# Autodesk Inventor assembly: asiyunit
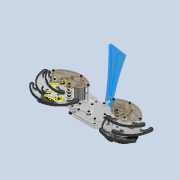
[picture p0: Inventor's stored thumbnail of the model, 180x180]
Saved by Autodesk Inventor 2020.4 (Build 244396000, 396)
## iProperties
Created: 2021-02-23
Part Number: asiyunit
Document SubType Name: Assembly
Designer: AA19065
Mass: 835.935 g
Surface Area: 3123.14 cm^2
Volume: 276.7 cm^3
Density: 3.02108 g/cm^3
Author: AA19065
## Documents named in this file (24)
- C:\Users\happy\OneDrive\ドキュメント\賢一ファイル\SRDC\試作10-2\アセンブリ\脚ユニット.iam
- C:\Users\happy\OneDrive\ドキュメント\賢一ファイル\SRDC\試作10-2\アセンブリ\前足.iam
- C:\Users\happy\OneDrive\ドキュメント\賢一ファイル\SRDC\試作10-2\アセンブリ\M-前足.iam
- C:\Users\happy\OneDrive\ドキュメント\賢一ファイル\SRDC\試作10-2\フレーム\脚中間フレーム内v2.ipt
- C:\Users\happy\OneDrive\ドキュメント\賢一ファイル\SRDC\試作10-2\フレーム\脚中間フレーム外v2.ipt
- C:\Users\happy\OneDrive\ドキュメント\賢一ファイル\SRDC\試作10-2\スペーサ\5mm.ipt
- C:\Users\happy\OneDrive\ドキュメント\賢一ファイル\SRDC\試作10-2\ねじ\m3皿ネジ5 (1).ipt
- C:\Users\happy\OneDrive\ドキュメント\賢一ファイル\SRDC\試作10-2\フレーム\アンノーン後.ipt
- C:\Users\happy\OneDrive\ドキュメント\賢一ファイル\SRDC\試作10-2\フレーム\アンノーン前.ipt
- C:\Users\happy\OneDrive\ドキュメント\賢一ファイル\SRDC\試作10-2\スペーサ\12mm.ipt
- C:\Users\happy\OneDrive\ドキュメント\賢一ファイル\SRDC\試作10-2\ねじ\M3ボタンボルト8.ipt
- C:\Users\happy\OneDrive\ドキュメント\賢一ファイル\SRDC\試作10-2\フレーム\heiko-ue.ipt
- C:\Users\happy\OneDrive\ドキュメント\賢一ファイル\SRDC\試作10-2\フレーム\hieko-sita.ipt
- C:\Users\happy\OneDrive\ドキュメント\賢一ファイル\SRDC\試作10-2\軸受け\オイレスw3f6-8a.ipt
- C:\Users\happy\OneDrive\ドキュメント\賢一ファイル\SRDC\試作10-2\軸受け\オイレスw1.5f6-8n.ipt
- C:\Users\happy\OneDrive\ドキュメント\賢一ファイル\SRDC\試作10-2\ねじ\ワッシャ3-8  0.5.ipt
- C:\Users\happy\OneDrive\ドキュメント\賢一ファイル\SRDC\試作10-2\スペーサ\18mm.ipt
- C:\Users\happy\OneDrive\ドキュメント\賢一ファイル\SRDC\試作10-2\アセンブリ\タミヤダンパー1.iam
- C:\Users\happy\OneDrive\ドキュメント\賢一ファイル\SRDC\試作10-2\スペーサ\8mm.ipt
- C:\Users\happy\OneDrive\ドキュメント\賢一ファイル\SRDC\試作10-2\ねじ\M3ボタンボルト20.ipt
- C:\Users\happy\OneDrive\ドキュメント\賢一ファイル\SRDC\試作10-2\ウィング\ウィング土台.ipt
- C:\Users\happy\OneDrive\ドキュメント\賢一ファイル\SRDC\試作10-2\ウィング\wing.ipt
- C:\Users\happy\OneDrive\ドキュメント\賢一ファイル\SRDC\試作10-2\ウィング\ウィングおさえ.ipt
- C:\Users\happy\OneDrive\ドキュメント\賢一ファイル\SRDC\試作10-2\ねじ\M3ボタンボルト12.ipt
## Components (69 placed, 23 different names)
1. 前足:1 [sub-assembly] — 挿入:48, 挿入:50, 挿入:54, 挿入:62, 挿入:70
2. M-前足:1 [sub-assembly] — 挿入:33, 挿入:61, 挿入:69
3. 脚中間フレーム内v2:1 — 挿入:1, 挿入:2, 挿入:3, 挿入:4, 挿入:7, 挿入:8, 挿入:9, 挿入:10, 挿入:11, 挿入:12, 挿入:13, 挿入:14, 挿入:15, 挿入:16, 挿入:21, 挿入:22, 挿入:23, 挿入:24, 挿入:25, 挿入:26, メイト:5, メイト:6, 挿入:63, 挿入:64, メイト:9
4. 脚中間フレーム外v2:1 — 挿入:5, 挿入:6, 挿入:17, 挿入:18, 挿入:19, 挿入:20, メイト:2, メイト:7, メイト:8
5. 5mm:1 — 挿入:1, 挿入:5, メイト:3
6. 5mm:2 — 挿入:4, 挿入:6
7. 5mm:3 — 挿入:2
8. 5mm:4 — 挿入:3
9. m3皿ネジ5 (1):1 — 挿入:7
10. m3皿ネジ5 (1):2 — 挿入:8
11. m3皿ネジ5 (1):3 — 挿入:9
12. m3皿ネジ5 (1):4 — 挿入:11
13. m3皿ネジ5 (1):5 — 挿入:12
14. m3皿ネジ5 (1):6 — 挿入:13
15. m3皿ネジ5 (1):7 — 挿入:14
16. m3皿ネジ5 (1):8 — 挿入:10
17. m3皿ネジ5 (1):9 — 挿入:15
18. m3皿ネジ5 (1):10 — 挿入:16
19. m3皿ネジ5 (1):11 — 挿入:20
20. m3皿ネジ5 (1):12 — 挿入:19
21. m3皿ネジ5 (1):13 — 挿入:18
22. m3皿ネジ5 (1):14 — 挿入:17
23. アンノーン後:1 — 挿入:29, 挿入:30, 挿入:37, 挿入:38, 挿入:39
24. アンノーン前:1 — 挿入:31, 挿入:32, 挿入:34, 挿入:35, 挿入:36
25. 12mm:1 — 挿入:26, 挿入:32
26. 12mm:2 — 挿入:24, 挿入:31
27. 12mm:3 — 挿入:25, メイト:1
28. 12mm:4 — 挿入:23, 挿入:29
29. 12mm:5 — 挿入:22, 挿入:33
30. 12mm:6 — 挿入:21, 挿入:30
31. M3ボタンボルト8:1 — 挿入:39
32. M3ボタンボルト8:2 — 挿入:38
33. M3ボタンボルト8:3 — 挿入:36
34. M3ボタンボルト8:4 — 挿入:37
35. M3ボタンボルト8:5 — 挿入:34
36. M3ボタンボルト8:6 — 挿入:35
37. heiko-ue:1 — 挿入:46, 挿入:49, メイト:2
38. hieko-sita:1 — 挿入:41, 挿入:51
39. オイレスw3f6-8a:1 — 挿入:41, メイト:1
40. オイレスw3f6-8a:3 — 挿入:49, メイト:3
41. 5mm:5 — 挿入:46, 挿入:47, 挿入:53
42. オイレスw3f6-8a:4 — 挿入:47, 挿入:48
43. オイレスw1.5f6-8n:1 — 挿入:50, 挿入:51
44. M3ボタンボルト8:7 — 挿入:52
45. ワッシャ3-8  0.5:1 — 挿入:52, 挿入:53
46. 18mm:1 — 挿入:54, 挿入:58, 挿入:71
47. M3ボタンボルト8:8
48. ワッシャ3-8  0.5:2 — 挿入:71
49. M3ボタンボルト8:9
50. ワッシャ3-8  0.5:3 — 挿入:58
51. タミヤダンパー1:1 [sub-assembly] — メイト:5, 挿入:61, 挿入:66, 挿入:68
52. タミヤダンパー1:2 [sub-assembly] — メイト:6, 挿入:62, 挿入:65, 挿入:67
53. 8mm:1 — 挿入:63
54. 8mm:2 — 挿入:64
55. M3ボタンボルト20:1 — 挿入:65
56. M3ボタンボルト20:2 — 挿入:66
57. M3ボタンボルト8:10 — 挿入:68
58. M3ボタンボルト8:11 — 挿入:67
59. M3ボタンボルト8:12 — 挿入:69
60. M3ボタンボルト8:13 — 挿入:70
61. ウィング土台:1 — メイト:7, メイト:8, メイト:9, 挿入:72, 挿入:73, 挿入:79, 挿入:80
62. 8mm:3 — 挿入:72, 挿入:74, 挿入:75
63. 8mm:4 — 挿入:73, 挿入:76
64. wing:1 — 挿入:74
65. ウィングおさえ:1 — 挿入:75, 挿入:76, 挿入:77, 挿入:78
66. M3ボタンボルト12:1 — 挿入:79
67. M3ボタンボルト12:2 — 挿入:78
68. M3ボタンボルト12:3 — 挿入:77
69. M3ボタンボルト12:4 — 挿入:80
## Relationships (78: Insert 70, Mate 8)
- 挿入:1 [Insert]: 脚中間フレーム内v2:1 ↔ 5mm:1
- 挿入:2 [Insert]: 脚中間フレーム内v2:1 ↔ 5mm:3
- 挿入:3 [Insert]: 脚中間フレーム内v2:1 ↔ 5mm:4
- 挿入:4 [Insert]: 脚中間フレーム内v2:1 ↔ 5mm:2
- 挿入:5 [Insert]: 脚中間フレーム外v2:1 ↔ 5mm:1
- 挿入:6 [Insert]: 脚中間フレーム外v2:1 ↔ 5mm:2
- 挿入:7 [Insert]: 脚中間フレーム内v2:1 ↔ m3皿ネジ5 (1):1
- 挿入:8 [Insert]: 脚中間フレーム内v2:1 ↔ m3皿ネジ5 (1):2
- 挿入:9 [Insert]: 脚中間フレーム内v2:1 ↔ m3皿ネジ5 (1):3
- 挿入:10 [Insert]: 脚中間フレーム内v2:1 ↔ m3皿ネジ5 (1):8
- 挿入:11 [Insert]: 脚中間フレーム内v2:1 ↔ m3皿ネジ5 (1):4
- 挿入:12 [Insert]: 脚中間フレーム内v2:1 ↔ m3皿ネジ5 (1):5
- 挿入:13 [Insert]: 脚中間フレーム内v2:1 ↔ m3皿ネジ5 (1):6
- 挿入:14 [Insert]: 脚中間フレーム内v2:1 ↔ m3皿ネジ5 (1):7
- 挿入:15 [Insert]: 脚中間フレーム内v2:1 ↔ m3皿ネジ5 (1):9
- 挿入:16 [Insert]: 脚中間フレーム内v2:1 ↔ m3皿ネジ5 (1):10
- 挿入:17 [Insert]: 脚中間フレーム外v2:1 ↔ m3皿ネジ5 (1):14
- 挿入:18 [Insert]: 脚中間フレーム外v2:1 ↔ m3皿ネジ5 (1):13
- 挿入:19 [Insert]: 脚中間フレーム外v2:1 ↔ m3皿ネジ5 (1):12
- 挿入:20 [Insert]: 脚中間フレーム外v2:1 ↔ m3皿ネジ5 (1):11
- 挿入:21 [Insert]: 脚中間フレーム内v2:1 ↔ 12mm:6
- 挿入:22 [Insert]: 脚中間フレーム内v2:1 ↔ 12mm:5
- 挿入:23 [Insert]: 脚中間フレーム内v2:1 ↔ 12mm:4
- 挿入:24 [Insert]: 脚中間フレーム内v2:1 ↔ 12mm:2
- 挿入:25 [Insert]: 脚中間フレーム内v2:1 ↔ 12mm:3
- 挿入:26 [Insert]: 脚中間フレーム内v2:1 ↔ 12mm:1
- 挿入:29 [Insert]: アンノーン後:1 ↔ 12mm:4
- 挿入:30 [Insert]: アンノーン後:1 ↔ 12mm:6
- 挿入:31 [Insert]: アンノーン前:1 ↔ 12mm:2
- 挿入:32 [Insert]: アンノーン前:1 ↔ 12mm:1
- 挿入:33 [Insert]: M-前足:1 ↔ 12mm:5
- 挿入:34 [Insert]: アンノーン前:1 ↔ M3ボタンボルト8:5
- 挿入:35 [Insert]: アンノーン前:1 ↔ M3ボタンボルト8:6
- 挿入:36 [Insert]: アンノーン前:1 ↔ M3ボタンボルト8:3
- 挿入:37 [Insert]: アンノーン後:1 ↔ M3ボタンボルト8:4
- 挿入:38 [Insert]: アンノーン後:1 ↔ M3ボタンボルト8:2
- 挿入:39 [Insert]: アンノーン後:1 ↔ M3ボタンボルト8:1
- 挿入:41 [Insert]: hieko-sita:1 ↔ オイレスw3f6-8a:1
- メイト:1 [Mate]: 12mm:3 ↔ オイレスw3f6-8a:1
- 挿入:46 [Insert]: heiko-ue:1 ↔ 5mm:5
- 挿入:47 [Insert] (1 mm): 5mm:5 ↔ オイレスw3f6-8a:4
- 挿入:48 [Insert]: 前足:1 ↔ オイレスw3f6-8a:4
- 挿入:49 [Insert]: heiko-ue:1 ↔ オイレスw3f6-8a:3
- メイト:2 [Mate]: 脚中間フレーム外v2:1 ↔ heiko-ue:1
- 挿入:50 [Insert]: 前足:1 ↔ オイレスw1.5f6-8n:1
- 挿入:51 [Insert]: hieko-sita:1 ↔ オイレスw1.5f6-8n:1
- メイト:3 [Mate]: 5mm:1 ↔ オイレスw3f6-8a:3
- 挿入:52 [Insert]: M3ボタンボルト8:7 ↔ ワッシャ3-8  0.5:1
- 挿入:53 [Insert]: 5mm:5 ↔ ワッシャ3-8  0.5:1
- 挿入:54 [Insert] (-3.5 mm): 前足:1 ↔ 18mm:1
- [Insert]: M3ボタンボルト8:8 ↔ ワッシャ3-8  0.5:2
- [Insert]: M3ボタンボルト8:9 ↔ ワッシャ3-8  0.5:3
- 挿入:58 [Insert]: 18mm:1 ↔ ワッシャ3-8  0.5:3
- メイト:5 [Mate]: 脚中間フレーム内v2:1 ↔ タミヤダンパー1:1
- メイト:6 [Mate]: 脚中間フレーム内v2:1 ↔ タミヤダンパー1:2
- 挿入:61 [Insert]: M-前足:1 ↔ タミヤダンパー1:1
- 挿入:62 [Insert]: 前足:1 ↔ タミヤダンパー1:2
- 挿入:63 [Insert]: 脚中間フレーム内v2:1 ↔ 8mm:1
- 挿入:64 [Insert]: 脚中間フレーム内v2:1 ↔ 8mm:2
- 挿入:65 [Insert]: タミヤダンパー1:2 ↔ M3ボタンボルト20:1
- 挿入:66 [Insert]: タミヤダンパー1:1 ↔ M3ボタンボルト20:2
- 挿入:67 [Insert]: タミヤダンパー1:2 ↔ M3ボタンボルト8:11
- 挿入:68 [Insert]: タミヤダンパー1:1 ↔ M3ボタンボルト8:10
- 挿入:69 [Insert]: M-前足:1 ↔ M3ボタンボルト8:12
- 挿入:70 [Insert]: 前足:1 ↔ M3ボタンボルト8:13
- 挿入:71 [Insert]: 18mm:1 ↔ ワッシャ3-8  0.5:2
- メイト:7 [Mate]: 脚中間フレーム外v2:1 ↔ ウィング土台:1
- メイト:8 [Mate]: 脚中間フレーム外v2:1 ↔ ウィング土台:1
- メイト:9 [Mate]: 脚中間フレーム内v2:1 ↔ ウィング土台:1
- 挿入:72 [Insert]: ウィング土台:1 ↔ 8mm:3
- 挿入:73 [Insert]: ウィング土台:1 ↔ 8mm:4
- 挿入:74 [Insert]: 8mm:3 ↔ wing:1
- 挿入:75 [Insert]: 8mm:3 ↔ ウィングおさえ:1
- 挿入:76 [Insert]: 8mm:4 ↔ ウィングおさえ:1
- 挿入:77 [Insert]: ウィングおさえ:1 ↔ M3ボタンボルト12:3
- 挿入:78 [Insert]: ウィングおさえ:1 ↔ M3ボタンボルト12:2
- 挿入:79 [Insert]: ウィング土台:1 ↔ M3ボタンボルト12:1
- 挿入:80 [Insert]: ウィング土台:1 ↔ M3ボタンボルト12:4
## Named parameters: d58_d55 = 0 mm, d59_d55 = 0 mm
